# Autodesk Inventor assembly: ZAxisBed
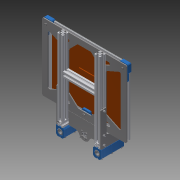
[picture p0: Inventor's stored thumbnail of the model, 180x180]
Saved by Autodesk Inventor 2015 SP1 (Build 190203100, 203)
## iProperties
Created: 2015-01-21
Part Number: ZAxisBed
Document SubType Name: Assembly
Designer: Jack
Mass: 2277.03 g
Surface Area: 6915.31 cm^2
Volume: 775.989 cm^3
Density: 2.93435 g/cm^3
Author: Jack
Title: Bed + Z Carriage
## Documents named in this file (27)
- C:\Users\Jack\ownCloud\Projects\CrossBot\InventorModel\ZAxis\ZAxisBed.iam
- C:\Users\Jack\ownCloud\Projects\CrossBot\InventorModel\Hardware\Bearing\BearingLinear\BearingLinearLMU10.ipt
- C:\Users\Jack\ownCloud\Projects\CrossBot\InventorModel\ZAxis\ZAxisCarriageRight.ipt
- C:\Users\Jack\ownCloud\Projects\CrossBot\InventorModel\ZAxis\ZAxisCarriageLeft.ipt
- C:\Users\Jack\ownCloud\Projects\CrossBot\InventorModel\HeatBed\Ultibots230x290\UltibotsBed230x290.iam
- C:\Users\Jack\ownCloud\Projects\CrossBot\InventorModel\ZAxis\ZAxisFrameVertical.ipt
- C:\Users\Jack\ownCloud\Projects\CrossBot\InventorModel\ZAxis\ZBedSupportExtrusion.ipt
- C:\Users\Jack\ownCloud\Projects\CrossBot\InventorModel\ZAxis\ZBedPlate.ipt
- C:\Users\Jack\ownCloud\Projects\CrossBot\InventorModel\HeatBed\BedClipUltiBots.ipt
- C:\Users\Jack\ownCloud\Projects\CrossBot\InventorModel\HeatBed\BedClipUltiBotsMirrored.ipt
- C:\Users\Jack\ownCloud\Projects\CrossBot\InventorModel\Hardware\Nuts\Nut3.ipt
- C:\Users\Jack\ownCloud\Projects\CrossBot\InventorModel\ZAxis\ZBedSupportLateral.ipt
- C:\Users\Jack\ownCloud\Projects\CrossBot\InventorModel\ZAxis\ZBedSupportPlate.ipt
- C:\Users\Jack\ownCloud\Projects\CrossBot\InventorModel\ZAxis\ZAxisNutMountMetal.ipt
- C:\Users\Jack\ownCloud\Projects\CrossBot\InventorModel\Hardware\BoltWashers\BoltWasher3\BoltWasher3x24.iam
- C:\Users\Jack\ownCloud\Projects\CrossBot\InventorModel\Hardware\BoltWashers\BoltWasher4\BoltWasher4x10.iam
- C:\Users\Jack\ownCloud\Projects\CrossBot\InventorModel\Hardware\Bolts\FHS\FHS4\FHS4x12.ipt
- C:\Users\Jack\ownCloud\Projects\CrossBot\InventorModel\Hardware\BoltWashers\BoltWasher3\BoltWasher3x16.iam
- C:\Users\Jack\ownCloud\Projects\CrossBot\InventorModel\Hardware\Wahsers\M3Washer.ipt
- C:\Users\Jack\ownCloud\Projects\CrossBot\InventorModel\HeatBed\BedClipUltiBotsMiddle.ipt
- C:\Users\Jack\ownCloud\Projects\CrossBot\InventorModel\Hardware\ZDrive\ZACMENut.ipt
- C:\Users\Jack\ownCloud\Projects\CrossBot\InventorModel\Hardware\BoltWashers\BoltWasher4\BoltWasher4x8.iam
- C:\Users\Jack\ownCloud\Projects\CrossBot\InventorModel\Hardware\Bolts\BlindExtrusionScrew\BlindExtrusionScrew5\M5x20BlindScrew.ipt
- C:\Users\Jack\ownCloud\Projects\CrossBot\InventorModel\Hardware\Nuts\ExtrusionNuts\ExtrusionNutHNKK5_4.ipt
- C:\Users\Jack\ownCloud\Projects\CrossBot\InventorModel\Hardware\Bolts\SHCS\SHCS4\SHCS4x10.ipt
- C:\Users\Jack\ownCloud\Projects\CrossBot\InventorModel\Hardware\Nuts\Nut4.ipt
- C:\Users\Jack\ownCloud\Projects\CrossBot\InventorModel\Hardware\Bolts\FHS\FHS4\FHS4x8.ipt
## Components (94 placed, 26 different names)
1. BedClipUltiBotsMirrored:1 — Mate:274, Angle:42, Mate:276, Mate:277, Mate:280
2. SHCS4x10:1 — Mate:279, Mate:282, Mate:285
3. SHCS4x10:2 — Mate:278, Mate:281, Mate:287
4. SHCS4x10:3 — Mate:277, Mate:280, Mate:283
5. Nut4:1 — Mate:283, Mate:284
6. Nut4:2 — Mate:285, Mate:286
7. Nut4:3 — Mate:287, Mate:288
8. ExtrusionNutHNKK5_4:19 — Mate:293, Angle:43, Mate:298
9. ExtrusionNutHNKK5_4:20 — Mate:294, Angle:46, Mate:297
10. ExtrusionNutHNKK5_4:21 — Mate:295, Angle:45, Mate:300
11. ExtrusionNutHNKK5_4:22 — Mate:296, Angle:44, Mate:299
12. FHS4x8:1 — Mate:291, Flush:39, Mate:294
13. FHS4x8:2 — Mate:290, Flush:37, Mate:296
14. FHS4x8:3 — Mate:292, Flush:38, Mate:295
15. FHS4x8:4 — Mate:289, Flush:36, Mate:293
16. BedClipUltiBotsMiddle:1 — Mate:197, Angle:25, Mate:275, Mate:279, Mate:282
17. BedClipUltiBots:1 — Mate:273, Mate:278, Mate:281
18. ZBedPlate:1 — Mate:76, Flush:23, Flush:34, Flush:35, Mate:197, Mate:273, Mate:274, Angle:42, Mate:275, Mate:276, Mate:284, Mate:286, Mate:288, Mate:289, Mate:290, Mate:291, Mate:292, Flush:36, Flush:37, Flush:38, Flush:39
19. UltibotsBed230x290:1 [sub-assembly] — Angle:25
20. ZAxisFrameVertical:1 — Mate:75, Flush:18, Flush:19, Mate:82, Flush:28, Flush:29, Mate:86, Mate:90, Mate:156, Mate:157, Mate:158, Angle:32, Angle:33, Mate:244, Mate:245, Angle:36, Mate:259, Angle:40, Angle:41, Mate:267, Mate:268, Mate:272
21. ZAxisFrameVertical:2 — Mate:74, Flush:17, Flush:20, Mate:78, Mate:80, Flush:26, Flush:30, Mate:84, Mate:153, Mate:154, Mate:155, Angle:34, Angle:35, Mate:248, Mate:249, Angle:37, Mate:260, Angle:38, Mate:262, Angle:39, Mate:264, Mate:271
22. ZBedSupportExtrusion:1 — Mate:74, Flush:17, Flush:20, Flush:22, Flush:32, Flush:34, Mate:229, Angle:26, Mate:231, Angle:28, Mate:235, Angle:29, Mate:237, Mate:270, Angle:44, Angle:45, Mate:299, Mate:300
23. ZBedSupportExtrusion:2 — Mate:75, Flush:18, Flush:19, Mate:76, Mate:77, Flush:23, Mate:83, Flush:31, Flush:33, Mate:88, Mate:228, Angle:27, Mate:233, Angle:30, Angle:31, Mate:246, Mate:247, Mate:269, Angle:43, Angle:46, Mate:297, Mate:298
24. ZBedSupportLateral:1 — Mate:77, Flush:22, Mate:83, Flush:31, Flush:35, Mate:226, Mate:227
25. ExtrusionNutHNKK5_4:2 — Mate:230, Angle:26, Mate:231
26. ExtrusionNutHNKK5_4:3 — Mate:232, Angle:27, Mate:233
27. BoltWasher4x8:1 [sub-assembly] — Mate:222, Mate:225, Mate:230
28. BoltWasher4x8:2 [sub-assembly] — Mate:223, Mate:224, Mate:232
29. ZAxisNutMountMetal:1 — Mate:88, Mate:89, Mate:90, Mate:192, Mate:193, Mate:195, Mate:210, Mate:211, Mate:212, Mate:213, Mate:214, Mate:215, Mate:216, Mate:222, Mate:223, Mate:224, Mate:225
30. ZACMENut:2 — Mate:215, Mate:216, Mate:217, Mate:218, Mate:219, Mate:220, Mate:221
31. BoltWasher3x16:1 [sub-assembly] — Mate:194, Mate:198, Mate:213, Mate:218
32. BoltWasher3x16:3 [sub-assembly] — Mate:190, Mate:199, Mate:212, Mate:219
33. BoltWasher3x16:2 [sub-assembly] — Mate:191, Mate:200, Mate:214, Mate:217, Mate:220
34. BoltWasher3x16:4 [sub-assembly] — Mate:210, Mate:221
35. Nut3:10
36. M3Washer:4 — Mate:211
37. M3Washer:1 — Mate:190, Mate:193, Mate:202
38. Nut3:8 — Mate:199, Mate:202
39. Nut3:9 — Mate:198, Mate:203
40. M3Washer:3 — Mate:194, Mate:195, Mate:203
41. Nut3:7 — Mate:200, Mate:201
42. M3Washer:2 — Mate:191, Mate:192, Mate:201
43. ExtrusionNutHNKK5_4:18 — Mate:266, Angle:41, Mate:267
44. ExtrusionNutHNKK5_4:14 — Mate:257, Angle:36, Mate:259
45. ExtrusionNutHNKK5_4:17 — Mate:265, Angle:40, Mate:268
46. FHS4x12:1 — Mate:152, Mate:156, Mate:265
47. FHS4x12:2 — Mate:151, Mate:157, Mate:257
48. FHS4x12:3 — Mate:150, Mate:158, Mate:266
49. BearingLinearLMU10:3 — Mate:37, Flush:16
50. BearingLinearLMU10:2 — Mate:42
51. ZAxisCarriageRight:1 — Mate:37, Flush:16, Angle:5, Angle:6, Angle:7, Mate:62, Mate:63, Mate:64, Flush:27, Mate:82, Flush:28, Flush:29, Mate:87, Mate:125, Mate:126, Mate:127, Mate:128, Mate:129, Mate:130, Mate:150, Mate:151, Mate:152
52. ExtrusionNutHNKK5_4:15 — Mate:261, Angle:38, Mate:262
53. ExtrusionNutHNKK5_4:13 — Mate:256, Angle:37, Mate:260
54. ExtrusionNutHNKK5_4:16 — Mate:263, Angle:39, Mate:264
55. FHS4x12:6 — Mate:149, Mate:155, Mate:263
56. FHS4x12:5 — Mate:148, Mate:154, Mate:256
57. FHS4x12:4 — Mate:147, Mate:153, Mate:261
58. ZAxisCarriageLeft:1 — Mate:36, Flush:15, Angle:8, Angle:9, Angle:10, Mate:65, Mate:66, Mate:67, Mate:78, Flush:24, Mate:79, Flush:25, Mate:80, Flush:26, Flush:27, Flush:30, Mate:85, Mate:119, Mate:120, Mate:121, Mate:122, Mate:123, Mate:124, Mate:147, Mate:148, Mate:149
59. BearingLinearLMU10:4 — Mate:36, Flush:15
60. BearingLinearLMU10:1 — Mate:42
61. M5x20BlindScrew:1 — Mate:226, Mate:229
62. M5x20BlindScrew:2 — Mate:227, Mate:228
63. M5x20BlindScrew:3 — Mate:269, Mate:272
64. M5x20BlindScrew:4 — Mate:270, Mate:271
65. ExtrusionNutHNKK5_4:12 — Mate:234, Angle:28, Mate:235
66. ExtrusionNutHNKK5_4:1 — Mate:236, Angle:29, Mate:237
67. ExtrusionNutHNKK5_4:4 — Mate:238, Angle:35, Mate:248
68. ExtrusionNutHNKK5_4:5 — Mate:239, Angle:34, Mate:249
69. BoltWasher4x10:2 [sub-assembly] — Mate:133, Mate:134, Mate:238
70. BoltWasher4x10:1 [sub-assembly] — Mate:131, Mate:132, Mate:239
71. BoltWasher4x10:3 [sub-assembly] — Mate:135, Mate:136, Mate:236
72. BoltWasher4x10:4 [sub-assembly] — Mate:137, Mate:138, Mate:234
73. ZBedSupportPlate:1 — Mate:84, Flush:32, Mate:85, Mate:131, Mate:132, Mate:133, Mate:134, Mate:135, Mate:136, Mate:137, Mate:138
74. ExtrusionNutHNKK5_4:9 — Mate:243, Angle:33, Mate:244
75. ExtrusionNutHNKK5_4:6 — Mate:242, Angle:32, Mate:245
76. ExtrusionNutHNKK5_4:7 — Mate:241, Angle:31, Mate:246
77. ExtrusionNutHNKK5_4:10 — Mate:240, Angle:30, Mate:247
78. BoltWasher4x10:7 [sub-assembly] — Mate:141, Mate:143, Mate:240
79. BoltWasher4x10:8 [sub-assembly] — Mate:140, Mate:144, Mate:241
80. BoltWasher4x10:5 [sub-assembly] — Mate:139, Mate:145, Mate:242
81. BoltWasher4x10:6 [sub-assembly] — Mate:142, Mate:146, Mate:243
82. ZBedSupportPlate:2 — Mate:86, Mate:87, Flush:33, Mate:89, Mate:139, Mate:140, Mate:141, Mate:142, Mate:143, Mate:144, Mate:145, Mate:146
83. BoltWasher3x24:5 [sub-assembly] — Mate:127, Mate:128, Mate:252
84. Nut3:3 — Angle:7, Mate:64, Mate:252
85. Nut3:1 — Angle:6, Mate:63, Mate:251
86. BoltWasher3x24:4 [sub-assembly] — Mate:126, Mate:129, Mate:251
87. BoltWasher3x24:6 [sub-assembly] — Mate:125, Mate:130, Mate:250
88. Nut3:2 — Angle:5, Mate:62, Mate:250
89. Nut3:6 — Angle:8, Mate:65, Mate:253
90. BoltWasher3x24:2 [sub-assembly] — Mate:119, Mate:124, Mate:253
91. Nut3:5 — Angle:9, Mate:66, Mate:254
92. BoltWasher3x24:3 [sub-assembly] — Mate:120, Mate:123, Mate:254
93. BoltWasher3x24:1 [sub-assembly] — Mate:121, Mate:122, Mate:255
94. Nut3:4 — Angle:10, Mate:67, Mate:255
## Relationships (234: Mate 176, Flush 29, Angle 29)
- [Mate]: ZAxisCarriageLeft:1 ↔ BearingLinearLMU10:1
- [Mate]: BearingLinearLMU10:2 ↔ ZAxisCarriageRight:1
- [Flush]: BearingLinearLMU10:2 ↔ ZAxisCarriageRight:1
- [Flush]: ZAxisCarriageLeft:1 ↔ BearingLinearLMU10:1
- [Flush]: ZAxisCarriageLeft:1 ↔ BearingLinearLMU10:4
- [Flush]: BearingLinearLMU10:3 ↔ ZAxisCarriageRight:1
- [Flush]: ZAxisCarriageRight:1 ↔ ZAxisCarriageLeft:1
- [Mate] (2 mm): BedClipUltiBots:1 ↔ ZBedPlate:1
- [Angle] (0 deg): BedClipUltiBots:1 ↔ ZBedPlate:1
- [Mate]: BedClipUltiBots:1 ↔ UltibotsBed230x290:1
- [Mate]: BedClipUltiBots:1 ↔ UltibotsBed230x290:1
- Mate:36: ZAxisCarriageLeft:1 ↔ BearingLinearLMU10:4
- Flush:15: ZAxisCarriageLeft:1 ↔ BearingLinearLMU10:4
- Mate:37: BearingLinearLMU10:3 ↔ ZAxisCarriageRight:1
- Flush:16: BearingLinearLMU10:3 ↔ ZAxisCarriageRight:1
- Mate:42 (130 mm): BearingLinearLMU10:2 ↔ BearingLinearLMU10:1
- Angle:5 (0 deg): ZAxisCarriageRight:1 ↔ Nut3:2
- Angle:6 (0 deg): ZAxisCarriageRight:1 ↔ Nut3:1
- Angle:7 (0 deg): ZAxisCarriageRight:1 ↔ Nut3:3
- Angle:8 (0 deg): ZAxisCarriageLeft:1 ↔ Nut3:6
- Angle:9 (0 deg): ZAxisCarriageLeft:1 ↔ Nut3:5
- Angle:10 (0 deg): ZAxisCarriageLeft:1 ↔ Nut3:4
- Mate:62: ZAxisCarriageRight:1 ↔ Nut3:2
- Mate:63: ZAxisCarriageRight:1 ↔ Nut3:1
- Mate:64: ZAxisCarriageRight:1 ↔ Nut3:3
- Mate:65: ZAxisCarriageLeft:1 ↔ Nut3:6
- Mate:66: ZAxisCarriageLeft:1 ↔ Nut3:5
- Mate:67: ZAxisCarriageLeft:1 ↔ Nut3:4
- Mate:74: ZAxisFrameVertical:2 ↔ ZBedSupportExtrusion:1
- Flush:17: ZAxisFrameVertical:2 ↔ ZBedSupportExtrusion:1
- Mate:75: ZAxisFrameVertical:1 ↔ ZBedSupportExtrusion:2
- Flush:18: ZAxisFrameVertical:1 ↔ ZBedSupportExtrusion:2
- Flush:19: ZAxisFrameVertical:1 ↔ ZBedSupportExtrusion:2
- Flush:20: ZAxisFrameVertical:2 ↔ ZBedSupportExtrusion:1
- Mate:76: ZBedPlate:1 ↔ ZBedSupportExtrusion:2
- Mate:77: ZBedSupportExtrusion:2 ↔ ZBedSupportLateral:1
- Flush:22: ZBedSupportExtrusion:1 ↔ ZBedSupportLateral:1
- Flush:23 (-73 mm): ZBedPlate:1 ↔ ZBedSupportExtrusion:2
- Mate:78: ZAxisFrameVertical:2 ↔ ZAxisCarriageLeft:1
- Flush:24: ZAxisCarriageLeft:1
- Mate:79: ZAxisCarriageLeft:1
- Flush:25: ZAxisCarriageLeft:1
- Mate:80: ZAxisFrameVertical:2 ↔ ZAxisCarriageLeft:1
- Flush:26 (4 mm): ZAxisFrameVertical:2 ↔ ZAxisCarriageLeft:1
- Flush:27: ZAxisCarriageRight:1 ↔ ZAxisCarriageLeft:1
- Mate:82: ZAxisFrameVertical:1 ↔ ZAxisCarriageRight:1
- Flush:28 (4 mm): ZAxisFrameVertical:1 ↔ ZAxisCarriageRight:1
- Flush:29: ZAxisFrameVertical:1 ↔ ZAxisCarriageRight:1
- Flush:30: ZAxisFrameVertical:2 ↔ ZAxisCarriageLeft:1
- Mate:83: ZBedSupportExtrusion:2 ↔ ZBedSupportLateral:1
- Flush:31: ZBedSupportExtrusion:2 ↔ ZBedSupportLateral:1
- Mate:84: ZAxisFrameVertical:2 ↔ ZBedSupportPlate:1
- Flush:32: ZBedSupportExtrusion:1 ↔ ZBedSupportPlate:1
- Mate:85: ZAxisCarriageLeft:1 ↔ ZBedSupportPlate:1
- Mate:86: ZAxisFrameVertical:1 ↔ ZBedSupportPlate:2
- Mate:87: ZAxisCarriageRight:1 ↔ ZBedSupportPlate:2
- Flush:33: ZBedSupportExtrusion:2 ↔ ZBedSupportPlate:2
- Flush:34: ZBedPlate:1 ↔ ZBedSupportExtrusion:1
- Flush:35 (108.25 mm): ZBedPlate:1 ↔ ZBedSupportLateral:1
- Mate:88: ZBedSupportExtrusion:2 ↔ ZAxisNutMountMetal:1
- Mate:89: ZAxisNutMountMetal:1 ↔ ZBedSupportPlate:2
- Mate:90: ZAxisFrameVertical:1 ↔ ZAxisNutMountMetal:1
- Mate:119: ZAxisCarriageLeft:1 ↔ BoltWasher3x24:2
- Mate:120: ZAxisCarriageLeft:1 ↔ BoltWasher3x24:3
- Mate:121: ZAxisCarriageLeft:1 ↔ BoltWasher3x24:1
- Mate:122: ZAxisCarriageLeft:1 ↔ BoltWasher3x24:1
- Mate:123: ZAxisCarriageLeft:1 ↔ BoltWasher3x24:3
- Mate:124: ZAxisCarriageLeft:1 ↔ BoltWasher3x24:2
- Mate:125: ZAxisCarriageRight:1 ↔ BoltWasher3x24:6
- Mate:126: ZAxisCarriageRight:1 ↔ BoltWasher3x24:4
- Mate:127: ZAxisCarriageRight:1 ↔ BoltWasher3x24:5
- Mate:128: ZAxisCarriageRight:1 ↔ BoltWasher3x24:5
- Mate:129: ZAxisCarriageRight:1 ↔ BoltWasher3x24:4
- Mate:130: ZAxisCarriageRight:1 ↔ BoltWasher3x24:6
- Mate:131: BoltWasher4x10:1 ↔ ZBedSupportPlate:1
- Mate:132: BoltWasher4x10:1 ↔ ZBedSupportPlate:1
- Mate:133: BoltWasher4x10:2 ↔ ZBedSupportPlate:1
- Mate:134: BoltWasher4x10:2 ↔ ZBedSupportPlate:1
- Mate:135: BoltWasher4x10:3 ↔ ZBedSupportPlate:1
- Mate:136: BoltWasher4x10:3 ↔ ZBedSupportPlate:1
- Mate:137: BoltWasher4x10:4 ↔ ZBedSupportPlate:1
- Mate:138: BoltWasher4x10:4 ↔ ZBedSupportPlate:1
- Mate:139: BoltWasher4x10:5 ↔ ZBedSupportPlate:2
- Mate:140: BoltWasher4x10:8 ↔ ZBedSupportPlate:2
- Mate:141: BoltWasher4x10:7 ↔ ZBedSupportPlate:2
- Mate:142: BoltWasher4x10:6 ↔ ZBedSupportPlate:2
- Mate:143: BoltWasher4x10:7 ↔ ZBedSupportPlate:2
- Mate:144: BoltWasher4x10:8 ↔ ZBedSupportPlate:2
- Mate:145: BoltWasher4x10:5 ↔ ZBedSupportPlate:2
- Mate:146: BoltWasher4x10:6 ↔ ZBedSupportPlate:2
- Mate:147: FHS4x12:4 ↔ ZAxisCarriageLeft:1
- Mate:148: FHS4x12:5 ↔ ZAxisCarriageLeft:1
- Mate:149: FHS4x12:6 ↔ ZAxisCarriageLeft:1
- Mate:150: FHS4x12:3 ↔ ZAxisCarriageRight:1
- Mate:151: FHS4x12:2 ↔ ZAxisCarriageRight:1
- Mate:152: FHS4x12:1 ↔ ZAxisCarriageRight:1
- Mate:153 (0.5 mm): ZAxisFrameVertical:2 ↔ FHS4x12:4
- Mate:154 (0.5 mm): ZAxisFrameVertical:2 ↔ FHS4x12:5
- Mate:155 (0.5 mm): ZAxisFrameVertical:2 ↔ FHS4x12:6
- Mate:156 (0.5 mm): ZAxisFrameVertical:1 ↔ FHS4x12:1
- Mate:157 (0.5 mm): ZAxisFrameVertical:1 ↔ FHS4x12:2
- Mate:158 (0.5 mm): ZAxisFrameVertical:1 ↔ FHS4x12:3
- Mate:190: BoltWasher3x16:3 ↔ M3Washer:1
- Mate:191: BoltWasher3x16:2 ↔ M3Washer:2
- Mate:192: ZAxisNutMountMetal:1 ↔ M3Washer:2
- Mate:193: ZAxisNutMountMetal:1 ↔ M3Washer:1
- Mate:194: BoltWasher3x16:1 ↔ M3Washer:3
- Mate:195: ZAxisNutMountMetal:1 ↔ M3Washer:3
- Mate:197 (2 mm): BedClipUltiBotsMiddle:1 ↔ ZBedPlate:1
- Angle:25 (0 deg): BedClipUltiBotsMiddle:1 ↔ UltibotsBed230x290:1
- Mate:198: BoltWasher3x16:1 ↔ Nut3:9
- Mate:199: BoltWasher3x16:3 ↔ Nut3:8
- Mate:200: BoltWasher3x16:2 ↔ Nut3:7
- Mate:201: Nut3:7 ↔ M3Washer:2
- Mate:202: M3Washer:1 ↔ Nut3:8
- Mate:203: Nut3:9 ↔ M3Washer:3
- [Mate]: BoltWasher3x16:4 ↔ M3Washer:4
- [Mate]: BoltWasher3x16:4 ↔ Nut3:10
- [Mate]: Nut3:10 ↔ M3Washer:4
- Mate:210: ZAxisNutMountMetal:1 ↔ BoltWasher3x16:4
- Mate:211: ZAxisNutMountMetal:1 ↔ M3Washer:4
- Mate:212: ZAxisNutMountMetal:1 ↔ BoltWasher3x16:3
- Mate:213: ZAxisNutMountMetal:1 ↔ BoltWasher3x16:1
- Mate:214: ZAxisNutMountMetal:1 ↔ BoltWasher3x16:2
- Mate:215: ZAxisNutMountMetal:1 ↔ ZACMENut:2
- Mate:216: ZAxisNutMountMetal:1 ↔ ZACMENut:2
- Mate:217: ZACMENut:2 ↔ BoltWasher3x16:2
- Mate:218: ZACMENut:2 ↔ BoltWasher3x16:1
- Mate:219: ZACMENut:2 ↔ BoltWasher3x16:3
- Mate:220: ZACMENut:2 ↔ BoltWasher3x16:2
- Mate:221: ZACMENut:2 ↔ BoltWasher3x16:4
- Mate:222: BoltWasher4x8:1 ↔ ZAxisNutMountMetal:1
- Mate:223: BoltWasher4x8:2 ↔ ZAxisNutMountMetal:1
- Mate:224: BoltWasher4x8:2 ↔ ZAxisNutMountMetal:1
- Mate:225: BoltWasher4x8:1 ↔ ZAxisNutMountMetal:1
- Mate:226: ZBedSupportLateral:1 ↔ M5x20BlindScrew:1
- Mate:227: ZBedSupportLateral:1 ↔ M5x20BlindScrew:2
- Mate:228: ZBedSupportExtrusion:2 ↔ M5x20BlindScrew:2
- Mate:229: ZBedSupportExtrusion:1 ↔ M5x20BlindScrew:1
- Mate:230: ExtrusionNutHNKK5_4:2 ↔ BoltWasher4x8:1
- Angle:26 (0 deg): ZBedSupportExtrusion:1 ↔ ExtrusionNutHNKK5_4:2
- Mate:231: ZBedSupportExtrusion:1 ↔ ExtrusionNutHNKK5_4:2
- Mate:232: ExtrusionNutHNKK5_4:3 ↔ BoltWasher4x8:2
- Angle:27 (0 deg): ZBedSupportExtrusion:2 ↔ ExtrusionNutHNKK5_4:3
- Mate:233: ZBedSupportExtrusion:2 ↔ ExtrusionNutHNKK5_4:3
- Mate:234: ExtrusionNutHNKK5_4:12 ↔ BoltWasher4x10:4
- Angle:28 (0 deg): ZBedSupportExtrusion:1 ↔ ExtrusionNutHNKK5_4:12
- Mate:235: ZBedSupportExtrusion:1 ↔ ExtrusionNutHNKK5_4:12
- Mate:236: ExtrusionNutHNKK5_4:1 ↔ BoltWasher4x10:3
- Angle:29 (0 deg): ZBedSupportExtrusion:1 ↔ ExtrusionNutHNKK5_4:1
- Mate:237: ZBedSupportExtrusion:1 ↔ ExtrusionNutHNKK5_4:1
- Mate:238: ExtrusionNutHNKK5_4:4 ↔ BoltWasher4x10:2
- Mate:239: ExtrusionNutHNKK5_4:5 ↔ BoltWasher4x10:1
- Mate:240: ExtrusionNutHNKK5_4:10 ↔ BoltWasher4x10:7
- Mate:241: ExtrusionNutHNKK5_4:7 ↔ BoltWasher4x10:8
- Mate:242: ExtrusionNutHNKK5_4:6 ↔ BoltWasher4x10:5
- Mate:243: ExtrusionNutHNKK5_4:9 ↔ BoltWasher4x10:6
- Angle:30 (0 deg): ZBedSupportExtrusion:2 ↔ ExtrusionNutHNKK5_4:10
- Angle:31 (0 deg): ZBedSupportExtrusion:2 ↔ ExtrusionNutHNKK5_4:7
- Angle:32 (0 deg): ZAxisFrameVertical:1 ↔ ExtrusionNutHNKK5_4:6
- Angle:33 (0 deg): ZAxisFrameVertical:1 ↔ ExtrusionNutHNKK5_4:9
- Mate:244: ZAxisFrameVertical:1 ↔ ExtrusionNutHNKK5_4:9
- Mate:245: ZAxisFrameVertical:1 ↔ ExtrusionNutHNKK5_4:6
- Mate:246: ZBedSupportExtrusion:2 ↔ ExtrusionNutHNKK5_4:7
- Mate:247: ZBedSupportExtrusion:2 ↔ ExtrusionNutHNKK5_4:10
- Angle:34 (0 deg): ZAxisFrameVertical:2 ↔ ExtrusionNutHNKK5_4:5
- Angle:35 (0 deg): ZAxisFrameVertical:2 ↔ ExtrusionNutHNKK5_4:4
- Mate:248: ZAxisFrameVertical:2 ↔ ExtrusionNutHNKK5_4:4
- Mate:249: ZAxisFrameVertical:2 ↔ ExtrusionNutHNKK5_4:5
- Mate:250: BoltWasher3x24:6 ↔ Nut3:2
- Mate:251: Nut3:1 ↔ BoltWasher3x24:4
- Mate:252: BoltWasher3x24:5 ↔ Nut3:3
- Mate:253: Nut3:6 ↔ BoltWasher3x24:2
- Mate:254: Nut3:5 ↔ BoltWasher3x24:3
- Mate:255: BoltWasher3x24:1 ↔ Nut3:4
- Mate:256: ExtrusionNutHNKK5_4:13 ↔ FHS4x12:5
- Mate:257: ExtrusionNutHNKK5_4:14 ↔ FHS4x12:2
- Angle:36 (0 deg): ZAxisFrameVertical:1 ↔ ExtrusionNutHNKK5_4:14
- Angle:37 (0 deg): ZAxisFrameVertical:2 ↔ ExtrusionNutHNKK5_4:13
- Mate:259: ZAxisFrameVertical:1 ↔ ExtrusionNutHNKK5_4:14
- Mate:260: ZAxisFrameVertical:2 ↔ ExtrusionNutHNKK5_4:13
- Mate:261: ExtrusionNutHNKK5_4:15 ↔ FHS4x12:4
- Angle:38 (0 deg): ZAxisFrameVertical:2 ↔ ExtrusionNutHNKK5_4:15
- Mate:262: ZAxisFrameVertical:2 ↔ ExtrusionNutHNKK5_4:15
- Mate:263: ExtrusionNutHNKK5_4:16 ↔ FHS4x12:6
- Angle:39 (0 deg): ZAxisFrameVertical:2 ↔ ExtrusionNutHNKK5_4:16
- Mate:264: ZAxisFrameVertical:2 ↔ ExtrusionNutHNKK5_4:16
- Mate:265: ExtrusionNutHNKK5_4:17 ↔ FHS4x12:1
- Mate:266: ExtrusionNutHNKK5_4:18 ↔ FHS4x12:3
- Angle:40 (0 deg): ZAxisFrameVertical:1 ↔ ExtrusionNutHNKK5_4:17
- Angle:41 (0 deg): ZAxisFrameVertical:1 ↔ ExtrusionNutHNKK5_4:18
- Mate:267: ZAxisFrameVertical:1 ↔ ExtrusionNutHNKK5_4:18
- Mate:268: ZAxisFrameVertical:1 ↔ ExtrusionNutHNKK5_4:17
- Mate:269: ZBedSupportExtrusion:2 ↔ M5x20BlindScrew:3
- Mate:270: ZBedSupportExtrusion:1 ↔ M5x20BlindScrew:4
- Mate:271: ZAxisFrameVertical:2 ↔ M5x20BlindScrew:4
- Mate:272: ZAxisFrameVertical:1 ↔ M5x20BlindScrew:3
- Mate:273: BedClipUltiBots:1 ↔ ZBedPlate:1
- Mate:274: BedClipUltiBotsMirrored:1 ↔ ZBedPlate:1
- Angle:42 (0 deg): BedClipUltiBotsMirrored:1 ↔ ZBedPlate:1
- Mate:275: BedClipUltiBotsMiddle:1 ↔ ZBedPlate:1
- Mate:276 (2 mm): BedClipUltiBotsMirrored:1 ↔ ZBedPlate:1
- Mate:277: BedClipUltiBotsMirrored:1 ↔ SHCS4x10:3
- Mate:278: SHCS4x10:2 ↔ BedClipUltiBots:1
- Mate:279: SHCS4x10:1 ↔ BedClipUltiBotsMiddle:1
- Mate:280: BedClipUltiBotsMirrored:1 ↔ SHCS4x10:3
- Mate:281: SHCS4x10:2 ↔ BedClipUltiBots:1
- Mate:282: SHCS4x10:1 ↔ BedClipUltiBotsMiddle:1
- Mate:283: SHCS4x10:3 ↔ Nut4:1
- Mate:284: Nut4:1 ↔ ZBedPlate:1
- Mate:285: SHCS4x10:1 ↔ Nut4:2
- Mate:286: Nut4:2 ↔ ZBedPlate:1
- Mate:287: SHCS4x10:2 ↔ Nut4:3
- Mate:288: Nut4:3 ↔ ZBedPlate:1
- Mate:289: FHS4x8:4 ↔ ZBedPlate:1
- Mate:290: FHS4x8:2 ↔ ZBedPlate:1
- Mate:291: FHS4x8:1 ↔ ZBedPlate:1
- Mate:292: FHS4x8:3 ↔ ZBedPlate:1
- Flush:36: FHS4x8:4 ↔ ZBedPlate:1
- Flush:37: FHS4x8:2 ↔ ZBedPlate:1
- Flush:38: FHS4x8:3 ↔ ZBedPlate:1
- Flush:39: FHS4x8:1 ↔ ZBedPlate:1
- Mate:293: ExtrusionNutHNKK5_4:19 ↔ FHS4x8:4
- Mate:294: ExtrusionNutHNKK5_4:20 ↔ FHS4x8:1
- Mate:295: ExtrusionNutHNKK5_4:21 ↔ FHS4x8:3
- Mate:296: ExtrusionNutHNKK5_4:22 ↔ FHS4x8:2
- Angle:43 (0 deg): ExtrusionNutHNKK5_4:19 ↔ ZBedSupportExtrusion:2
- Angle:44 (0 deg): ExtrusionNutHNKK5_4:22 ↔ ZBedSupportExtrusion:1
- Angle:45 (0 deg): ExtrusionNutHNKK5_4:21 ↔ ZBedSupportExtrusion:1
- Angle:46 (0 deg): ExtrusionNutHNKK5_4:20 ↔ ZBedSupportExtrusion:2
- Mate:297: ExtrusionNutHNKK5_4:20 ↔ ZBedSupportExtrusion:2
- Mate:298: ExtrusionNutHNKK5_4:19 ↔ ZBedSupportExtrusion:2
- Mate:299: ExtrusionNutHNKK5_4:22 ↔ ZBedSupportExtrusion:1
- Mate:300: ExtrusionNutHNKK5_4:21 ↔ ZBedSupportExtrusion:1
## Named parameters: d373_d360 = 0 mm, d374_d365 = 0 mm, d375_d370 = 0 mm
